# Autodesk Inventor assembly: rack and pinion
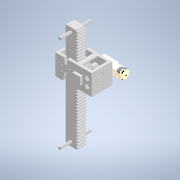
[picture p0: Inventor's stored thumbnail of the model, 180x180]
Saved by Autodesk Inventor 2020.1 (Build 241239000, 239)
## iProperties
Created: 2019-11-10
Part Number: rack and pinion
Document SubType Name: Assembly
Designer: amirs
Author: amirs
## Documents named in this file (9)
- C:\Users\amirs\Downloads\rack and pinion.iam
- C:\Users\amirs\Downloads\NewCasing.ipt
- C:\Users\amirs\Downloads\Rack.ipt
- C:\Users\amirs\Downloads\Pinion.ipt
- C:\Users\amirs\Downloads\Motor Shaft Extension.ipt
- C:\Users\amirs\Downloads\Solarbotics_GM9-Assem.iam
- C:\Users\amirs\Downloads\front delrin.ipt
- C:\Users\amirs\Downloads\delrin for sides.ipt
- C:\Users\amirs\OneDrive - UC San Diego\college\freshman year\MAE 3\robot\rack and pinion\stopper shaft.ipt
## Components (16 placed, 8 different names)
1. NewCasing:1 — Mate:1, Mate:2, Mate:3, Mate:14, Mate:25, Mate:26, Mate:27, Mate:29, Mate:30, Mate:31, Mate:32, Mate:33, Mate:34, Mate:35, Mate:36, Mate:37
2. Rack:1 — Mate:18, Mate:19, Mate:20, Mate:38
3. Rack:2 — Mate:21, Mate:22, Mate:23, Mate:39, Mate:40
4. Rack:3 — Mate:14, Mate:15, Mate:16, Mate:17, Mate:18, Mate:19, Mate:20, Mate:42
5. Rack:4 — Mate:15, Mate:16, Mate:17, Mate:21, Mate:22, Mate:23, Mate:41
6. Pinion:1 — Mate:8, Flush:2, Mate:9, Flush:3, Mate:10
7. Pinion:3 — Mate:6, Mate:8, Flush:2, Mate:11
8. Pinion:4 — Mate:9, Flush:3, Mate:10, Mate:11
9. Motor Shaft Extension:1 — Mate:4, Mate:5, Mate:6
10. Solarbotics_GM9-Assem:1 [sub-assembly] — Mate:1, Mate:2, Mate:3, Mate:4, Mate:5
11. front delrin:1 — Mate:31, Mate:32, Mate:33
12. front delrin:2 — Mate:34, Mate:35, Mate:36, Mate:38
13. delrin for sides:1 — Mate:25, Mate:26, Mate:27
14. delrin for sides:2 — Mate:29, Mate:30, Mate:37
15. stopper shaft:1 — Mate:39, Mate:42
16. stopper shaft:2 — Mate:40, Mate:41
## Relationships (39: Mate 37, Flush 2)
- Mate:1: NewCasing:1 ↔ Solarbotics_GM9-Assem:1
- Mate:2: NewCasing:1 ↔ Solarbotics_GM9-Assem:1
- Mate:3: NewCasing:1 ↔ Solarbotics_GM9-Assem:1
- Mate:4: Motor Shaft Extension:1 ↔ Solarbotics_GM9-Assem:1
- Mate:5: Motor Shaft Extension:1 ↔ Solarbotics_GM9-Assem:1
- Mate:6: Pinion:3 ↔ Motor Shaft Extension:1
- Mate:8: Pinion:1 ↔ Pinion:3
- Flush:2: Pinion:1 ↔ Pinion:3
- Mate:9: Pinion:1 ↔ Pinion:4
- Flush:3: Pinion:1 ↔ Pinion:4
- Mate:10: Pinion:1 ↔ Pinion:4
- Mate:11: Pinion:3 ↔ Pinion:4
- Mate:14 (1.27 mm): NewCasing:1 ↔ Rack:3
- Mate:15: Rack:3 ↔ Rack:4
- Mate:16: Rack:3 ↔ Rack:4
- Mate:17: Rack:3 ↔ Rack:4
- Mate:18: Rack:1 ↔ Rack:3
- Mate:19: Rack:1 ↔ Rack:3
- Mate:20: Rack:1 ↔ Rack:3
- Mate:21: Rack:2 ↔ Rack:4
- Mate:22: Rack:2 ↔ Rack:4
- Mate:23: Rack:2 ↔ Rack:4
- Mate:25: NewCasing:1 ↔ delrin for sides:1
- Mate:26: NewCasing:1 ↔ delrin for sides:1
- Mate:27: NewCasing:1 ↔ delrin for sides:1
- Mate:29: NewCasing:1 ↔ delrin for sides:2
- Mate:30: NewCasing:1 ↔ delrin for sides:2
- Mate:31: NewCasing:1 ↔ front delrin:1
- Mate:32: NewCasing:1 ↔ front delrin:1
- Mate:33: NewCasing:1 ↔ front delrin:1
- Mate:34: NewCasing:1 ↔ front delrin:2
- Mate:35: NewCasing:1 ↔ front delrin:2
- Mate:36: NewCasing:1 ↔ front delrin:2
- Mate:37: NewCasing:1 ↔ delrin for sides:2
- Mate:38 (0.6096 mm): Rack:1 ↔ front delrin:2
- Mate:39: Rack:2 ↔ stopper shaft:1
- Mate:40: Rack:2 ↔ stopper shaft:2
- Mate:41 (-38.1 mm): Rack:4 ↔ stopper shaft:2
- Mate:42 (-38.1 mm): Rack:3 ↔ stopper shaft:1
